# Autodesk Inventor assembly: shooter launcher
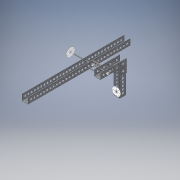
[picture p0: Inventor's stored thumbnail of the model, 180x180]
Saved by Autodesk Inventor 2017 (Build 210142000, 142)
## iProperties
Created: 2018-05-23
Part Number: shooter launcher
Document SubType Name: Assembly
Designer: User
Author: User
## Documents named in this file (9)
- C:\Robotics\CAD\2018-19_CAD\Offseason\shooter launcher.iam
- C:\Robotics\CAD\COTSParts\Actobotics\585 parts\585466Channel24in.ipt
- C:\Robotics\CAD\COTSParts\Actobotics\585 parts\585446Channel6in.ipt
- C:\Robotics\CAD\COTSParts\Actobotics\585 parts\585628FlatPattern90degreesA.ipt
- C:\Robotics\CAD\COTSParts\Tetrix\Hex standoff 2in.ipt
- C:\Robotics\CAD\COTSParts\Actobotics\634 parts\634088.25inDShaft8inLong.ipt
- C:\Robotics\CAD\COTSParts\Actobotics\615 parts\615106Sprocket.5inBore.25inPitch24Teeth.ipt
- C:\Robotics\CAD\COTSParts\Actobotics\535 parts\535198Bearing.25ID.5OD.ipt
- C:\Robotics\CAD\COTSParts\Actobotics\Collar.ipt
## Components (19 placed, 8 different names)
1. 585466Channel24in:1 — Flush:7, Mate:4, Flush:8, Mate:6, Mate:7, Mate:8, Mate:9
2. 585446Channel6in:1 — Mate:1, Flush:1, Flush:2, Mate:2, Flush:4, Mate:3, Flush:6, Flush:7, Insert:1, Insert:2, Insert:3, Insert:4, Mate:10, Mate:11, Mate:12, Mate:13
3. 585446Channel6in:2 — Mate:1, Flush:1, Flush:2, Flush:3, Flush:5, Flush:8
4. 585628FlatPattern90degreesA:1 — Mate:3, Flush:5, Flush:6
5. 585628FlatPattern90degreesA:2 — Mate:2, Flush:3, Flush:4
6. Hex standoff 2in:1 — Insert:2
7. Hex standoff 2in:2 — Insert:3, Mate:4
8. Hex standoff 2in:3 — Insert:1
9. 634088.25inDShaft8inLong:1 — Insert:4, Mate:5, Angle:1, Angle:2, Angle:3, Angle:4
10. 615106Sprocket.5inBore.25inPitch24Teeth:1 — Mate:5
11. 615106Sprocket.5inBore.25inPitch24Teeth:2
12. 535198Bearing.25ID.5OD:1 — Mate:8, Mate:9, Insert:7
13. 535198Bearing.25ID.5OD:2 — Mate:12, Mate:13, Insert:5
14. 535198Bearing.25ID.5OD:3 — Mate:10, Mate:11, Insert:6
15. 535198Bearing.25ID.5OD:4 — Mate:6, Mate:7, Insert:8
16. Collar:1 — Angle:2, Insert:6
17. Collar:2 — Insert:5, Angle:1
18. Collar:3 — Insert:7, Angle:3
19. Collar:4 — Insert:8, Angle:4
## Relationships (33: Mate 13, Flush 8, Insert 8, Angle 4)
- Mate:1: 585446Channel6in:1 ↔ 585446Channel6in:2
- Flush:1: 585446Channel6in:1 ↔ 585446Channel6in:2
- Flush:2: 585446Channel6in:1 ↔ 585446Channel6in:2
- Mate:2: 585446Channel6in:1 ↔ 585628FlatPattern90degreesA:2
- Flush:3: 585446Channel6in:2 ↔ 585628FlatPattern90degreesA:2
- Flush:4: 585446Channel6in:1 ↔ 585628FlatPattern90degreesA:2
- Mate:3: 585446Channel6in:1 ↔ 585628FlatPattern90degreesA:1
- Flush:5: 585446Channel6in:2 ↔ 585628FlatPattern90degreesA:1
- Flush:6: 585446Channel6in:1 ↔ 585628FlatPattern90degreesA:1
- Flush:7: 585466Channel24in:1 ↔ 585446Channel6in:1
- Insert:1: 585446Channel6in:1 ↔ Hex standoff 2in:3
- Insert:2: 585446Channel6in:1 ↔ Hex standoff 2in:1
- Insert:3: 585446Channel6in:1 ↔ Hex standoff 2in:2
- Mate:4: 585466Channel24in:1 ↔ Hex standoff 2in:2
- Flush:8 (114.3 mm): 585466Channel24in:1 ↔ 585446Channel6in:2
- Insert:4 (7.1882 mm): 585446Channel6in:1 ↔ 634088.25inDShaft8inLong:1
- Mate:5: 634088.25inDShaft8inLong:1 ↔ 615106Sprocket.5inBore.25inPitch24Teeth:1
- Mate:6: 585466Channel24in:1 ↔ 535198Bearing.25ID.5OD:4
- Mate:7: 585466Channel24in:1 ↔ 535198Bearing.25ID.5OD:4
- Mate:8: 585466Channel24in:1 ↔ 535198Bearing.25ID.5OD:1
- Mate:9: 585466Channel24in:1 ↔ 535198Bearing.25ID.5OD:1
- Mate:10: 585446Channel6in:1 ↔ 535198Bearing.25ID.5OD:3
- Mate:11: 585446Channel6in:1 ↔ 535198Bearing.25ID.5OD:3
- Mate:12: 585446Channel6in:1 ↔ 535198Bearing.25ID.5OD:2
- Mate:13: 585446Channel6in:1 ↔ 535198Bearing.25ID.5OD:2
- Insert:5: 535198Bearing.25ID.5OD:2 ↔ Collar:2
- Angle:1 (0 deg): 634088.25inDShaft8inLong:1 ↔ Collar:2
- Angle:2 (0 deg): 634088.25inDShaft8inLong:1 ↔ Collar:1
- Insert:6: 535198Bearing.25ID.5OD:3 ↔ Collar:1
- Insert:7: 535198Bearing.25ID.5OD:1 ↔ Collar:3
- Angle:3 (0 deg): 634088.25inDShaft8inLong:1 ↔ Collar:3
- Insert:8: 535198Bearing.25ID.5OD:4 ↔ Collar:4
- Angle:4 (0 deg): 634088.25inDShaft8inLong:1 ↔ Collar:4
